# Autodesk Inventor assembly: laser dichroic and beam steering subassy v2
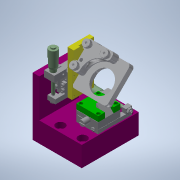
[picture p0: Inventor's stored thumbnail of the model, 180x180]
Saved by Autodesk Inventor 2022 (Build 260153000, 153)
## iProperties
Created: 2011-09-10
Part Number: laser dichroic and beam steering subassy v2
Document SubType Name: Assembly
Designer: betzige
Author: betzige
## Documents named in this file (8)
- G:\My Drive\OPM\2P-OPM_CAD\workspace\1P Laser Combiner\laser dichroic and beam steering subassy v2.iam
- G:\My Drive\OPM\2P-OPM_CAD\workspace\1P Laser Combiner\9061 micro translation stage 25 mm platform.iam
- G:\My Drive\OPM\2P-OPM_CAD\workspace\1P Laser Combiner\newfocus_9884_pint_size_corner_mount.iam
- G:\My Drive\OPM\2P-OPM_CAD\workspace\1P Laser Combiner\9354 micrometer 6p5 mm travel.ipt
- G:\My Drive\OPM\2P-OPM_CAD\workspace\1P Laser Combiner\MRA10-E02 right angle prism dielectric coat.ipt
- G:\My Drive\OPM\2P-OPM_CAD\workspace\1P Laser Combiner\prism to x stage mounting plate.ipt
- G:\My Drive\OPM\2P-OPM_CAD\workspace\1P Laser Combiner\mirror translation stage adapter.ipt
- G:\My Drive\OPM\2P-OPM_CAD\workspace\1P Laser Combiner\beam steering subassy mounting bracket.ipt
## Components (9 placed, 7 different names)
1. 9061 micro translation stage 25 mm platform:1 [sub-assembly] — Mate:14, Mate:15, Mate:16, Mate:17, Mate:18, Angle:2, Angle:3, Mate:27
2. newfocus_9884_pint_size_corner_mount:1 [sub-assembly] — Angle:1, Mate:23, Mate:24
3. 9354 micrometer 6p5 mm travel:1 — Mate:17, Mate:18
4. 9354 micrometer 6p5 mm travel:2 — Mate:4, Mate:5
5. 9061 micro translation stage 25 mm platform:2 [sub-assembly] — Mate:1, Mate:4, Mate:5, Mate:6, Mate:26, Mate:28, Mate:29
6. MRA10-E02 right angle prism dielectric coat:1 — Mate:6, Mate:7, Mate:8, Mate:9, Mate:10, Mate:11, Flush:1
7. prism to x stage mounting plate:1 — Mate:1, Mate:7, Mate:8, Mate:28, Mate:29
8. mirror translation stage adapter:1 — Angle:1, Mate:14, Mate:15, Mate:16, Mate:23, Mate:24
9. beam steering subassy mounting bracket:1 — Mate:26, Mate:27, Flush:1
## Relationships (24: Mate 20, Angle 3, Flush 1)
- Mate:1: 9061 micro translation stage 25 mm platform:2 ↔ prism to x stage mounting plate:1
- Mate:4: 9354 micrometer 6p5 mm travel:2 ↔ 9061 micro translation stage 25 mm platform:2
- Mate:5: 9354 micrometer 6p5 mm travel:2 ↔ 9061 micro translation stage 25 mm platform:2
- Mate:6: 9061 micro translation stage 25 mm platform:2 ↔ MRA10-E02 right angle prism dielectric coat:1
- Mate:7: MRA10-E02 right angle prism dielectric coat:1 ↔ prism to x stage mounting plate:1
- Mate:8: MRA10-E02 right angle prism dielectric coat:1 ↔ prism to x stage mounting plate:1
- Mate:9: MRA10-E02 right angle prism dielectric coat:1
- Mate:10: MRA10-E02 right angle prism dielectric coat:1
- Mate:11: MRA10-E02 right angle prism dielectric coat:1
- Angle:1 (0 deg): newfocus_9884_pint_size_corner_mount:1 ↔ mirror translation stage adapter:1
- Mate:14: 9061 micro translation stage 25 mm platform:1 ↔ mirror translation stage adapter:1
- Mate:15: 9061 micro translation stage 25 mm platform:1 ↔ mirror translation stage adapter:1
- Mate:16: 9061 micro translation stage 25 mm platform:1 ↔ mirror translation stage adapter:1
- Mate:17: 9061 micro translation stage 25 mm platform:1 ↔ 9354 micrometer 6p5 mm travel:1
- Mate:18: 9061 micro translation stage 25 mm platform:1 ↔ 9354 micrometer 6p5 mm travel:1
- Angle:2 (180 deg): 9061 micro translation stage 25 mm platform:1
- Angle:3 (180 deg): 9061 micro translation stage 25 mm platform:1
- Mate:23: newfocus_9884_pint_size_corner_mount:1 ↔ mirror translation stage adapter:1
- Mate:24: newfocus_9884_pint_size_corner_mount:1 ↔ mirror translation stage adapter:1
- Mate:26: 9061 micro translation stage 25 mm platform:2 ↔ beam steering subassy mounting bracket:1
- Mate:27: 9061 micro translation stage 25 mm platform:1 ↔ beam steering subassy mounting bracket:1
- Flush:1: MRA10-E02 right angle prism dielectric coat:1 ↔ beam steering subassy mounting bracket:1
- Mate:28: 9061 micro translation stage 25 mm platform:2 ↔ prism to x stage mounting plate:1
- Mate:29: 9061 micro translation stage 25 mm platform:2 ↔ prism to x stage mounting plate:1
